# Autodesk Inventor assembly: ZStopAssembly
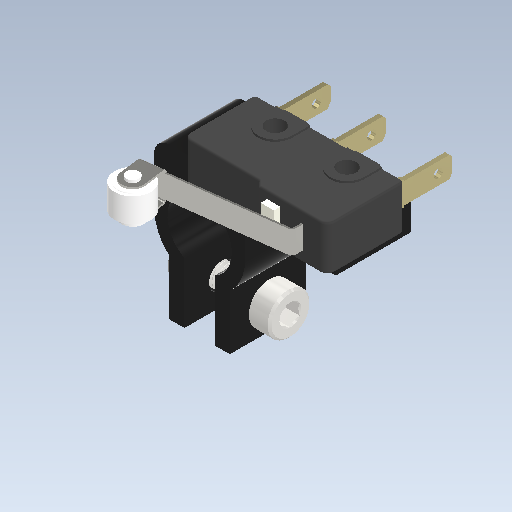
[picture p0: Inventor's stored thumbnail of the model, 512x512]
Saved by Autodesk Inventor 2020.2 (Build 242310000, 310)
## iProperties
Created: 2020-08-28
Part Number: ZStopAssembly
Document SubType Name: Assembly
Designer: JK
Author: JK
## Documents named in this file (5)
- C:\Users\JK\Documents\Inventor\Anet Upgrade\ZStopAssembly.iam
- C:\Users\JK\Documents\Inventor\Anet Upgrade\ZStopMount.ipt
- C:\Users\JK\Documents\Inventor\Anet Upgrade\EndStop.ipt
- C:\Users\JK\Documents\Inventor\Anet Upgrade\M3x10.ipt
- C:\Users\JK\Documents\Inventor\Anet Upgrade\M3Nut.ipt
## Components (4 placed, 4 different names)
1. ZStopMount:1 — Mate:3, Mate:5, Mate:6
2. EndStop:1
3. M3x10:1 — Mate:3, Mate:4, Mate:5
4. M3Nut:1 — Mate:4, Mate:6
## Relationships (6: Mate 6)
- [Mate]: ZStopMount:1 ↔ EndStop:1
- [Mate]: ZStopMount:1 ↔ EndStop:1
- Mate:3: ZStopMount:1 ↔ M3x10:1
- Mate:4: M3x10:1 ↔ M3Nut:1
- Mate:5: ZStopMount:1 ↔ M3x10:1
- Mate:6: ZStopMount:1 ↔ M3Nut:1
